# Autodesk Inventor assembly: ASY PNS FDS way3_1600
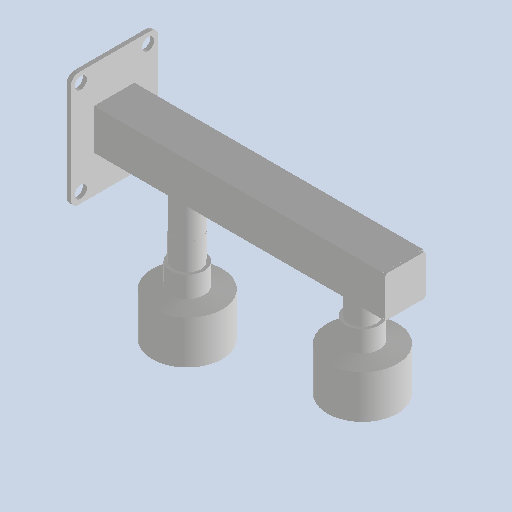
[picture p0: Inventor's stored thumbnail of the model, 512x512]
Saved by Autodesk Inventor 2025 (Build 290162010, 162A)
## iProperties
Created: 2025-07-02
Part Number: ASY PNS FDS way3_1600
Document SubType Name: Assembly
Designer: admin
Author: user
## Documents named in this file (7)
- C:\Users\pokla\Documents\Inventor\PNS2-Panaevsk\Filter D1000\filter-distribution-system 1000\ASY PNS FDS way3_1600.iam
- C:\Users\pokla\Documents\Inventor\PNS2-Panaevsk\Filter D1000\filter-distribution-system 1000\PNS 1663 FDS 1200 way tube 3.ipt
- C:\Users\pokla\Documents\Inventor\PNS2-Panaevsk\Filter D1000\filter-distribution-system 1000\PNS dummy filter element_1600.ipt
- C:\Users\pokla\Documents\Inventor\PNS2-Panaevsk\Filter D1000\filter-distribution-system 1000\PNS dummy pipe nippel_1600.ipt
- C:\Users\pokla\Documents\Inventor\PNS2-Panaevsk\Filter D1000\filter-distribution-system 1000\PNS 1687 FDS 1000 way tube 7.ipt
- C:\Users\pokla\Documents\Inventor\PNS2-Panaevsk\Filter D1000\filter-distribution-system 1000\PNS 1669 FDS 1000 FLANGE 3.ipt
- C:\Users\pokla\Documents\Inventor\PNS2-Panaevsk\Filter D1000\filter-distribution-system 1000\PNS 1666 FDS 1000 CUP 1.ipt
## Components (8 placed, 6 different names)
1. PNS 1663 FDS 1200 way tube 3.ipt:1 — Rigid:2, Rigid:5, Rigid:6, Rigid:7
2. PNS dummy filter element_1600.ipt:1 — Rigid:1
3. PNS dummy pipe nippel_1600.ipt:1 — Rigid:2, Rigid:1
4. PNS 1687 FDS 1000 way tube 7.ipt:1 — Rigid:5, Rigid:4
5. PNS dummy filter element_1600.ipt:2 — Rigid:3
6. PNS dummy pipe nippel_1600.ipt:2 — Rigid:4, Rigid:3
7. PNS 1669 FDS 1000 FLANGE 3.ipt:1 — Rigid:6
8. PNS 1666 FDS 1000 CUP 1.ipt:1 — Rigid:7
## Relationships (7: WeldJoint 7)
- Rigid:2 [WeldJoint]: PNS 1663 FDS 1200 way tube 3.ipt:1 ↔ PNS dummy pipe nippel_1600.ipt:1
- Rigid:1 [WeldJoint]: PNS dummy filter element_1600.ipt:1 ↔ PNS dummy pipe nippel_1600.ipt:1
- Rigid:5 [WeldJoint]: PNS 1663 FDS 1200 way tube 3.ipt:1 ↔ PNS 1687 FDS 1000 way tube 7.ipt:1
- Rigid:4 [WeldJoint]: PNS 1687 FDS 1000 way tube 7.ipt:1 ↔ PNS dummy pipe nippel_1600.ipt:2
- Rigid:3 [WeldJoint]: PNS dummy filter element_1600.ipt:2 ↔ PNS dummy pipe nippel_1600.ipt:2
- Rigid:6 [WeldJoint] (-3 mm): PNS 1663 FDS 1200 way tube 3.ipt:1 ↔ PNS 1669 FDS 1000 FLANGE 3.ipt:1
- Rigid:7 [WeldJoint]: PNS 1663 FDS 1200 way tube 3.ipt:1 ↔ PNS 1666 FDS 1000 CUP 1.ipt:1
